# Autodesk Inventor assembly: Zespół2
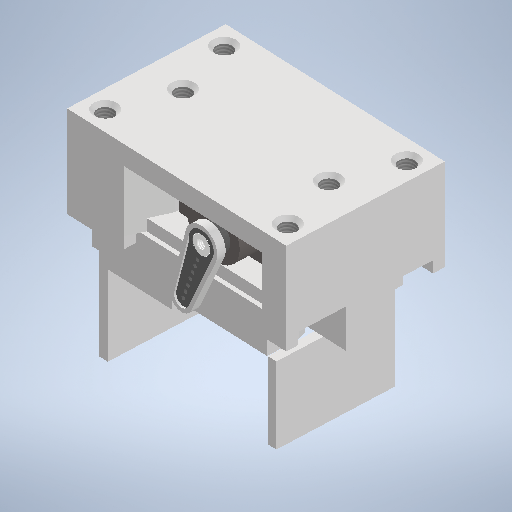
[picture p0: Inventor's stored thumbnail of the model, 512x512]
Saved by Autodesk Inventor 2025.2 (Build 292293000, 293)
## iProperties
Created: 2026-05-04
Part Number: Zespół2
Document SubType Name: Assembly
Designer: muszy
Author: muszy
## Documents named in this file (11)
- C:\Users\muszy\Documents\Robot_projekt\Gripper\Zespół2.iam
- C:\Users\muszy\Documents\Robot_projekt\Gripper\Podstawa.ipt
- C:\Users\muszy\Documents\falownik- step\falownik\M90S_ali\M90S_ali.iam
- C:\Users\muszy\Documents\Robot_projekt\Gripper\MG90S_arm01\MG90S_arm01\MG90S_arm01.ipt
- C:\Users\muszy\Documents\Robot_projekt\Gripper\podstawka.ipt
- C:\Users\muszy\Documents\Robot_projekt\Gripper\środek.ipt
- C:\Users\muszy\Documents\Robot_projekt\Gripper\slizg.ipt
- C:\Users\muszy\Documents\Robot_projekt\Gripper\chwyt.ipt
- C:\Users\muszy\Documents\Robot_projekt\Gripper\Zespół2\Design Accelerator\Przekładnie walcowe4.iam
- C:\Users\muszy\Documents\Robot_projekt\Gripper\slizg_serwo.ipt
- C:\Users\muszy\Documents\Robot_projekt\Gripper\adapter.ipt
## Components (11 placed, 10 different names)
1. Podstawa:1 — Zestawiające:1, Równoległe:1, Równoległe:2, Zestawiające:2, Zestawiające:3, Zestawiające:4, Zestawiające:5, Zestawiające:6, Zestawiające:9, przesuwne:1, Zestawiające:10, Zestawiające:11
2. M90S_ali:1 [sub-assembly] — Zestawiające:1, Równoległe:1, Obrotowe:1
3. MG90S_arm01:1 — Obrotowe:1, Sztywne:3
4. podstawka:1 — Równoległe:2, Zestawiające:2, Zestawiające:3
5. środek:1 — Zestawiające:4, Zestawiające:5, Zestawiające:6, Wstawiające:10
6. slizg:1 — Równoległe:3, Zestawiające:7, Zestawiające:8, Obrót/przesunięcie:1, Zestawiające:9, przesuwne:1
7. chwyt:1 — Równoległe:3, Zestawiające:7, Zestawiające:8
8. Przekładnie walcowe:1 [sub-assembly] — Wstawiające:10, Obrót/przesunięcie:1, Obrót/przesunięcie:2
9. slizg_serwo:1 — Zestawiające:10, Obrót/przesunięcie:2, Zestawiające:11, Zestawiające:12, Zestawiające:13, Zestawiające:14, Styczny:1
10. chwyt:2 — Zestawiające:12, Zestawiające:13, Zestawiające:14
11. adapter:1 — Sztywne:3, Styczny:1
## Relationships (24: Mate 14, Flush 3, RelateRotateTranslate 2, Insert 1, TranslationJoint 1, RevoluteJoint 1, WeldJoint 1, Tangent 1)
- Zestawiające:1 [Mate]: Podstawa:1 ↔ M90S_ali:1
- Równoległe:1 [Flush]: Podstawa:1 ↔ M90S_ali:1
- Równoległe:2 [Flush]: Podstawa:1 ↔ podstawka:1
- Zestawiające:2 [Mate]: Podstawa:1 ↔ podstawka:1
- Zestawiające:3 [Mate]: Podstawa:1 ↔ podstawka:1
- Zestawiające:4 [Mate]: Podstawa:1 ↔ środek:1
- Zestawiające:5 [Mate]: Podstawa:1 ↔ środek:1
- Zestawiające:6 [Mate]: Podstawa:1 ↔ środek:1
- Równoległe:3 [Flush]: slizg:1 ↔ chwyt:1
- Zestawiające:7 [Mate]: slizg:1 ↔ chwyt:1
- Zestawiające:8 [Mate]: slizg:1 ↔ chwyt:1
- Wstawiające:10 [Insert]: środek:1 ↔ Przekładnie walcowe:1
- Obrót/przesunięcie:1 [RelateRotateTranslate] (47.1239 mm): slizg:1 ↔ Przekładnie walcowe:1
- Zestawiające:9 [Mate]: Podstawa:1 ↔ slizg:1
- przesuwne:1 [TranslationJoint]: Podstawa:1 ↔ slizg:1
- Zestawiające:10 [Mate]: Podstawa:1 ↔ slizg_serwo:1
- Obrót/przesunięcie:2 [RelateRotateTranslate] (47.1239 mm): Przekładnie walcowe:1 ↔ slizg_serwo:1
- Zestawiające:11 [Mate] (0.1 mm): Podstawa:1 ↔ slizg_serwo:1
- Zestawiające:12 [Mate]: slizg_serwo:1 ↔ chwyt:2
- Zestawiające:13 [Mate]: slizg_serwo:1 ↔ chwyt:2
- Zestawiające:14 [Mate]: slizg_serwo:1 ↔ chwyt:2
- Obrotowe:1 [RevoluteJoint]: M90S_ali:1 ↔ MG90S_arm01:1
- Sztywne:3 [WeldJoint]: MG90S_arm01:1 ↔ adapter:1
- Styczny:1 [Tangent]: slizg_serwo:1 ↔ adapter:1
